# Autodesk Inventor assembly: ASY PNS 1600 Filter column D1000
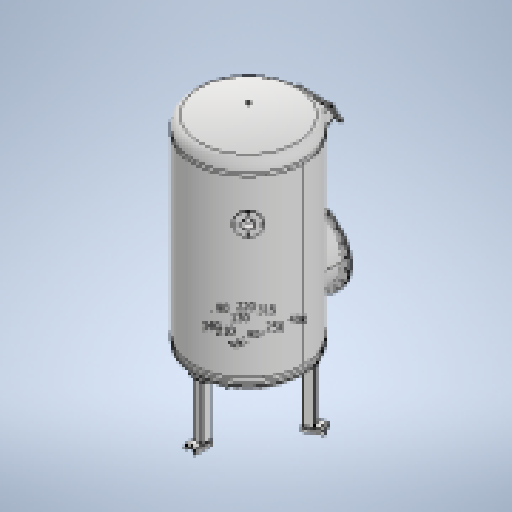
[picture p0: Inventor's stored thumbnail of the model, 512x512]
Saved by Autodesk Inventor 2025.3 (Build 293356030, 356C)
## iProperties
Created: 2025-02-13
Part Number: ASY PNS 1600 Filter column D1000
Document SubType Name: Assembly
Designer: pokla
Mass: 294380 g
Surface Area: 201489 cm^2
Volume: 65316.1 cm^3
Density: 4.50701 g/cm^3
allow_slope_adjustment: 0 ul
flow_configuration2: 1 ul
flow_direction: 2 ul
loss_method: 0 ul
radius: 45,500 mm
radius: 16,750 mm
Author: pokla
Revision Number: 3
## iProperties of the stored document MemberDocs/xS3xdvqv2Fs4urkfuOqhnp5u1Be
allow_slope_adjustment: 0 ul
flow_configuration2: 1 ul
flow_direction: 2 ul
loss_method: 0 ul
radius: 45,500 mm
Created: 2025-02-13
Part Number: ASY PNS 1600 Filter column D1000
Document SubType Name: Assembly
Designer: pokla
Mass: 294380 g
Surface Area: 201489 cm^2
Volume: 65316.1 cm^3
Density: 4.50701 g/cm^3
radius: 16,750 mm
Author: pokla
Revision Number: 3
## iProperties of the stored document MemberDocs/xVvj5wjhiIso5nm03Gzgds4hn2d
Created: 2025-02-13
Part Number: ASY PNS 1600 Filter column D1000
Document SubType Name: Assembly
Designer: pokla
Mass: 294380 g
Surface Area: 201489 cm^2
Volume: 65316.1 cm^3
Density: 4.50701 g/cm^3
allow_slope_adjustment: 0 ul
flow_configuration2: 1 ul
flow_direction: 2 ul
loss_method: 0 ul
radius: 45,500 mm
radius: 16,750 mm
Author: pokla
Revision Number: 3
## Documents named in this file (25)
- C:\Users\admin\Documents\Inventor\SLM-Salemal\ASY SLM 1600 Filter column D940.iam
- C:\Users\admin\Documents\Inventor\SLM-Salemal\PNS-612 accses hatch flangeipt.ipt
- C:\Users\admin\Documents\Inventor\SLM-Salemal\SLM 1601 DIM Filter column D940.ipt
- C:\Users\admin\Documents\Inventor\SLM-Salemal\PNS-611 accses hatch tube.ipt
- C:\Users\admin\Documents\Inventor\SLM-Salemal\PNS 1602 main Shell D1000.ipt
- C:\Users\admin\Documents\Inventor\SLM-Salemal\PNS 1604 dished head D1000.ipt
- C:\Users\admin\Documents\Inventor\SLM-Salemal\Fitting G1.ipt
- C:\Users\admin\Documents\Inventor\SLM-Salemal\ASY PNS 1690 Filter legs D1000.iam
- C:\Users\admin\Documents\Inventor\SLM-Salemal\PNS 1633 charging blind flange.ipt
- C:\Users\admin\Documents\Inventor\SLM-Salemal\ASY PNS 1610 charging hatch.iam
- C:\Users\admin\Documents\Inventor\SLM-Salemal\cc\JIS B 2312 90 Deg Long Elbow Steel 80A x Sch 40.ipt
- C:\Users\admin\Documents\Inventor\SLM-Salemal\ASY PNS 1650 filter-distribution-system 1000.iam
- C:\Users\admin\Documents\Inventor\SLM-Salemal\PNS 1612 FDS tube 2.ipt
- C:\Users\admin\Documents\Inventor\SLM-Salemal\PNS 1606 charging flange round.ipt
- C:\Users\admin\Documents\Inventor\SLM-Salemal\PNS 1613 FDS tube 3.ipt
- C:\Users\admin\Documents\Inventor\SLM-Salemal\PNS 1614 FDS tube 4.ipt
- C:\Users\admin\Documents\Inventor\SLM-Salemal\PNS 1615 FDS tube 5.ipt
- C:\Users\admin\Documents\Inventor\SLM-Salemal\ASY PNS 179 top funnel 1200 50-90_1000x90.iam
- C:\Users\admin\Documents\Inventor\SLM-Salemal\pallet jack dummy.ipt
- C:\Users\admin\Documents\Inventor\SLM-Salemal\SLM 1431 FDS flange DN90.ipt
- C:\Users\admin\Documents\Inventor\SLM-Salemal\SLM 1432 FDS free flange DN90.ipt
- C:\Users\admin\Documents\Inventor\SLM-Salemal\SLM 1671 charging tube 1.ipt
- C:\Users\admin\Documents\Inventor\SLM-Salemal\SLM 1672 charging tube 2.ipt
- C:\Users\admin\Documents\Inventor\SLM-Salemal\PNS 1607 charging flange rect.ipt
- C:\Users\admin\Documents\Inventor\SLM-Salemal\PNS 1607 charging flange cup.ipt
## Components (28 placed, 24 different names)
1. PNS 1601 DIM Filter column D1000.ipt:1
2. PNS 1602 main Shell D1000.ipt:1 — Rigid:10, Rigid:13, Rigid:14, Mate:1, Mate:2, Rigid:74, Rigid:80, Rigid:81
3. Fitting G1.ipt:1 — Rigid:15
4. PNS 1633 charging blind flange.ipt:2 — Rigid:67
5. ASY PNS 1650 filter-distribution-system 1000.iam:1 [sub-assembly] — Rotational:75
6. ASY PNS 179 top funnel 1200 50-90_1000x90:1 [sub-assembly] — Rotational:72
7. pallet jack dummy:1
8. PNS 1633 charging blind flange:5 — Rigid:77
9. PNS 1633 charging blind flange:6 — Rigid:78, Rotational:72
10. PNS 1604 dished head D1000.ipt:1 — Rigid:13, Rigid:75
11. Fitting G1.ipt:2
12. ASY PNS 1690 Filter legs D1000.iam:1 [sub-assembly] — Flush:2, Flush:3
13. JIS B 2312 90 Deg Long Elbow Steel 80A x Sch 40.ipt:1 — Rigid:68, Rigid:79
14. PNS 1613 FDS tube 3:1 — Rigid:67, Rigid:68, Flush:3
15. PNS 1614 FDS tube 4:1 — Rigid:79, Rigid:75, Rotational:71, Rotational:75
16. SLM 1431 FDS flange DN90:1 — Rigid:76
17. SLM 1432 FDS free flange DN90:1 — Rotational:71, Rigid:76
18. PNS-611 accses hatch tube.ipt:1 — Rigid:10, Rotational:74
19. PNS 1604 dished head D1000.ipt:2 — Rigid:14, Rigid:15, Mate:3
20. JIS B 2312 90 Deg Long Elbow Steel 80A x Sch 40.ipt:2 — Rigid:62, Rigid:73
21. PNS 1612 FDS tube 2:3 — Rigid:62, Rigid:78
22. PNS 1615 FDS tube 5:1 — Rigid:73, Rigid:74, Rigid:77
23. SLM 1672 charging tube 2:1 — Rigid:81, Rigid:82
24. SLM 1671 charging tube 1:1 — Rigid:80
25. PNS 1606 charging flange round:1 — Rigid:82, Rigid:83
26. PNS 1607 charging flange rect:1 — Rigid:83
27. PNS-612 accses hatch flangeipt.ipt:1 — Rotational:73, Rotational:74
28. ASY PNS 1610 charging hatch.iam:1 [sub-assembly] — Rotational:73
## Relationships (28: WeldJoint 18, RevoluteJoint 5, Mate 3, Flush 2)
- Rigid:10 [WeldJoint] (66 mm): PNS 1602 main Shell D1000.ipt:1 ↔ PNS-611 accses hatch tube.ipt:1
- Rigid:13 [WeldJoint]: PNS 1602 main Shell D1000.ipt:1 ↔ PNS 1604 dished head D1000.ipt:1
- Rigid:14 [WeldJoint]: PNS 1602 main Shell D1000.ipt:1 ↔ PNS 1604 dished head D1000.ipt:2
- Rigid:15 [WeldJoint]: Fitting G1.ipt:1 ↔ PNS 1604 dished head D1000.ipt:2
- Mate:1: PNS 1602 main Shell D1000.ipt:1
- Mate:2: PNS 1602 main Shell D1000.ipt:1
- Mate:3 (2300 mm): PNS 1604 dished head D1000.ipt:2
- Flush:2: ASY PNS 1690 Filter legs D1000.iam:1
- Rigid:62 [WeldJoint]: JIS B 2312 90 Deg Long Elbow Steel 80A x Sch 40.ipt:2 ↔ PNS 1612 FDS tube 2:3
- Rigid:67 [WeldJoint]: PNS 1633 charging blind flange.ipt:2 ↔ PNS 1613 FDS tube 3:1
- Rigid:68 [WeldJoint]: JIS B 2312 90 Deg Long Elbow Steel 80A x Sch 40.ipt:1 ↔ PNS 1613 FDS tube 3:1
- Rigid:79 [WeldJoint]: JIS B 2312 90 Deg Long Elbow Steel 80A x Sch 40.ipt:1 ↔ PNS 1614 FDS tube 4:1
- Rigid:73 [WeldJoint]: JIS B 2312 90 Deg Long Elbow Steel 80A x Sch 40.ipt:2 ↔ PNS 1615 FDS tube 5:1
- Rigid:74 [WeldJoint] (80 mm): PNS 1602 main Shell D1000.ipt:1 ↔ PNS 1615 FDS tube 5:1
- Rigid:75 [WeldJoint] (-50 mm): PNS 1604 dished head D1000.ipt:1 ↔ PNS 1614 FDS tube 4:1
- Flush:3: ASY PNS 1690 Filter legs D1000.iam:1 ↔ PNS 1613 FDS tube 3:1
- Rotational:71 [RevoluteJoint]: PNS 1614 FDS tube 4:1 ↔ SLM 1432 FDS free flange DN90:1
- Rigid:76 [WeldJoint]: SLM 1431 FDS flange DN90:1 ↔ SLM 1432 FDS free flange DN90:1
- Rigid:77 [WeldJoint]: PNS 1633 charging blind flange:5 ↔ PNS 1615 FDS tube 5:1
- Rigid:78 [WeldJoint]: PNS 1633 charging blind flange:6 ↔ PNS 1612 FDS tube 2:3
- Rotational:72 [RevoluteJoint]: ASY PNS 179 top funnel 1200 50-90_1000x90:1 ↔ PNS 1633 charging blind flange:6
- Rotational:73 [RevoluteJoint]: PNS-612 accses hatch flangeipt.ipt:1 ↔ ASY PNS 1610 charging hatch.iam:1
- Rotational:74 [RevoluteJoint]: PNS-611 accses hatch tube.ipt:1 ↔ PNS-612 accses hatch flangeipt.ipt:1
- Rotational:75 [RevoluteJoint]: ASY PNS 1650 filter-distribution-system 1000.iam:1 ↔ PNS 1614 FDS tube 4:1
- Rigid:80 [WeldJoint]: PNS 1602 main Shell D1000.ipt:1 ↔ SLM 1671 charging tube 1:1
- Rigid:81 [WeldJoint]: PNS 1602 main Shell D1000.ipt:1 ↔ SLM 1672 charging tube 2:1
- Rigid:82 [WeldJoint]: SLM 1672 charging tube 2:1 ↔ PNS 1606 charging flange round:1
- Rigid:83 [WeldJoint]: PNS 1606 charging flange round:1 ↔ PNS 1607 charging flange rect:1
